# Autodesk Inventor assembly: T
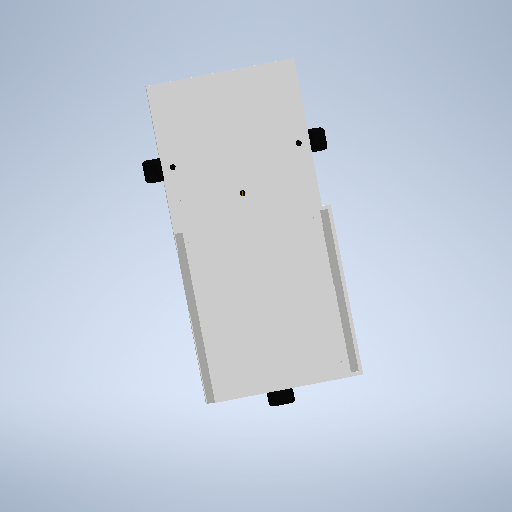
[picture p0: Inventor's stored thumbnail of the model, 512x512]
Saved by Autodesk Inventor 2025.3 (Build 293356000, 356)
## iProperties
Created: 2026-04-18
Part Number: T
Document SubType Name: Assembly
Designer: ksawe
Author: ksawe
## Documents named in this file (6)
- C:\Users\ksawe\OneDrive\Pulpit\Exomy v1\wersja3\T.iam
- C:\Users\ksawe\OneDrive\Pulpit\Exomy v1\wersja3\L.ipt
- C:\Users\ksawe\OneDrive\Pulpit\Exomy v1\wersja3\e.ipt
- C:\Users\ksawe\OneDrive\Pulpit\Exomy v1\wersja3\panel1.ipt
- C:\Users\ksawe\OneDrive\Pulpit\Exomy v1\wersja3\panel2.ipt
- C:\Users\ksawe\OneDrive\Pulpit\Exomy v1\wersja3\Box.ipt
## Components (5 placed, 5 different names)
1. L:1 — Mate:1, Mate:2, Mate:3, Mate:7, Mate:8, Mate:9, Mate:14
2. e:1 — Mate:1, Mate:2, Mate:3, Mate:4, Mate:5, Mate:6, Mate:14
3. panel1:1 — Mate:4, Mate:5, Mate:6, Mate:11
4. panel2:1 — Mate:7, Mate:8, Mate:9, Mate:10, Mate:12, Mate:13
5. Box:1 — Mate:10, Mate:11, Mate:12, Mate:13
## Relationships (14: Mate 14)
- Mate:1: L:1 ↔ e:1
- Mate:2: L:1 ↔ e:1
- Mate:3: L:1 ↔ e:1
- Mate:4: e:1 ↔ panel1:1
- Mate:5: e:1 ↔ panel1:1
- Mate:6: e:1 ↔ panel1:1
- Mate:7: L:1 ↔ panel2:1
- Mate:8: L:1 ↔ panel2:1
- Mate:9: L:1 ↔ panel2:1
- Mate:10: panel2:1 ↔ Box:1
- Mate:11: panel1:1 ↔ Box:1
- Mate:12: panel2:1 ↔ Box:1
- Mate:13: panel2:1 ↔ Box:1
- Mate:14: L:1 ↔ e:1
